# Autodesk Inventor assembly: Arm_Assembly
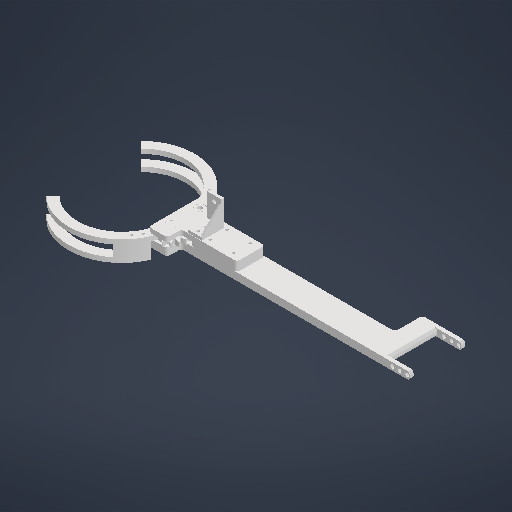
[picture p0: Inventor's stored thumbnail of the model, 512x512]
Saved by Autodesk Inventor 2026.1 (Build 301233020, 233B)
## iProperties
Created: 2025-10-28
Part Number: Arm_Assembly
Document SubType Name: Assembly
Designer: Garfieldcmix
Author: Garfieldcmix
## Documents named in this file (8)
- C:\Users\Garfieldcmix\git\KMITL-ComPro-Group-Work\models\manual-robot\Arm_Assembly.iam
- C:\Users\Garfieldcmix\git\KMITL-ComPro-Group-Work\models\manual-robot\Arm.ipt
- C:\Users\Garfieldcmix\git\KMITL-ComPro-Group-Work\models\manual-robot\Arm_Top.ipt
- C:\Users\Garfieldcmix\git\KMITL-ComPro-Group-Work\models\manual-robot\Left_Top_Gripper.ipt
- C:\Users\Garfieldcmix\git\KMITL-ComPro-Group-Work\models\manual-robot\Right_Top_Gripper.ipt
- C:\Users\Garfieldcmix\git\KMITL-ComPro-Group-Work\models\manual-robot\Servo_Holder.ipt
- C:\Users\Garfieldcmix\git\KMITL-ComPro-Group-Work\models\manual-robot\Left_Bottom_Gripper.ipt
- C:\Users\Garfieldcmix\git\KMITL-ComPro-Group-Work\models\manual-robot\Right_Bottom_Gripper.ipt
## Components (7 placed, 7 different names)
1. Arm:1 — Mate:1, Mate:2, Mate:3, Rotational:1, Rotational:2
2. Arm_Top:1 — Mate:1, Mate:2, Mate:3, Mate:4, Mate:5, Mate:6
3. Left_Top_Gripper:1 — Mate:10, Mate:11, Mate:12, Rotational:2, Rotation:1
4. Right_Top_Gripper:1 — Mate:7, Mate:8, Mate:9, Rotational:1, Rotation:1
5. Servo_Holder:1 — Mate:4, Mate:5, Mate:6
6. Left_Bottom_Gripper:1 — Mate:10, Mate:11, Mate:12
7. Right_Bottom_Gripper:1 — Mate:7, Mate:8, Mate:9
## Relationships (15: Mate 12, RevoluteJoint 2, RelateRotation 1)
- Mate:1: Arm:1 ↔ Arm_Top:1
- Mate:2: Arm:1 ↔ Arm_Top:1
- Mate:3: Arm:1 ↔ Arm_Top:1
- Mate:4: Arm_Top:1 ↔ Servo_Holder:1
- Mate:5: Arm_Top:1 ↔ Servo_Holder:1
- Mate:6: Arm_Top:1 ↔ Servo_Holder:1
- Mate:7: Right_Top_Gripper:1 ↔ Right_Bottom_Gripper:1
- Mate:8: Right_Top_Gripper:1 ↔ Right_Bottom_Gripper:1
- Mate:9: Right_Top_Gripper:1 ↔ Right_Bottom_Gripper:1
- Mate:10: Left_Top_Gripper:1 ↔ Left_Bottom_Gripper:1
- Mate:11: Left_Top_Gripper:1 ↔ Left_Bottom_Gripper:1
- Mate:12: Left_Top_Gripper:1 ↔ Left_Bottom_Gripper:1
- Rotational:1 [RevoluteJoint]: Arm:1 ↔ Right_Top_Gripper:1
- Rotational:2 [RevoluteJoint]: Arm:1 ↔ Left_Top_Gripper:1
- Rotation:1 [RelateRotation] (1 ul): Left_Top_Gripper:1 ↔ Right_Top_Gripper:1
